# Autodesk Inventor assembly: cat
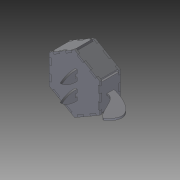
[picture p0: Inventor's stored thumbnail of the model, 180x180]
Saved by Autodesk Inventor 2015 (Build 190159000, 159)
## iProperties
Created: 2017-11-28
Part Number: cat
Document SubType Name: Assembly
Designer: Max
Author: Max
## Documents named in this file (8)
- C:\Users\Max\Dropbox\cat\cat.iam
- C:\Users\Max\Dropbox\cat\base.ipt
- C:\Users\Max\Dropbox\cat\cara.ipt
- C:\Users\Max\Dropbox\cat\lado.ipt
- C:\Users\Max\Dropbox\cat\cabeza.ipt
- C:\Users\Max\Dropbox\cat\oreja.ipt
- C:\Users\Max\Dropbox\cat\lado cola.ipt
- C:\Users\Max\Dropbox\cat\cola.ipt
## Components (11 placed, 7 different names)
1. base:1 — Flush:1, Mate:1, Mate:2, Flush:2, Mate:3, Mate:4, Flush:3, Mate:5, Mate:6, Flush:4, Mate:7, Mate:8, Flush:6, Mate:11, Mate:12, Mate:21
2. cara:1 — Flush:1, Mate:1, Mate:2, Flush:7, Mate:13, Mate:14
3. lado:1 — Flush:3, Mate:5, Mate:6
4. lado:3 — Flush:4, Mate:7, Mate:8
5. lado:5 — Flush:2, Mate:3, Mate:4
6. lado:7 — Flush:6, Mate:11, Mate:12
7. cabeza:1 — Flush:7, Mate:13, Mate:14, Mate:15, Mate:16, Mate:17, Mate:18, Mate:19, Mate:20, Flush:8, Mate:22
8. oreja:1 — Mate:18, Mate:19, Mate:20
9. oreja:2 — Mate:15, Mate:16, Mate:17
10. lado cola:1 — Flush:8, Mate:21, Mate:22, Mate:23, Mate:24
11. cola:1 — Mate:23, Mate:24
## Relationships (29: Mate 22, Flush 7)
- Flush:1: base:1 ↔ cara:1
- Mate:1: base:1 ↔ cara:1
- Mate:2: base:1 ↔ cara:1
- Flush:2: base:1 ↔ lado:5
- Mate:3: base:1 ↔ lado:5
- Mate:4: base:1 ↔ lado:5
- Flush:3: base:1 ↔ lado:1
- Mate:5: base:1 ↔ lado:1
- Mate:6: base:1 ↔ lado:1
- Flush:4: base:1 ↔ lado:3
- Mate:7: base:1 ↔ lado:3
- Mate:8: base:1 ↔ lado:3
- Flush:6: base:1 ↔ lado:7
- Mate:11: base:1 ↔ lado:7
- Mate:12: base:1 ↔ lado:7
- Flush:7: cara:1 ↔ cabeza:1
- Mate:13: cara:1 ↔ cabeza:1
- Mate:14: cara:1 ↔ cabeza:1
- Mate:15: cabeza:1 ↔ oreja:2
- Mate:16: cabeza:1 ↔ oreja:2
- Mate:17: cabeza:1 ↔ oreja:2
- Mate:18: cabeza:1 ↔ oreja:1
- Mate:19: cabeza:1 ↔ oreja:1
- Mate:20: cabeza:1 ↔ oreja:1
- Flush:8: cabeza:1 ↔ lado cola:1
- Mate:21: base:1 ↔ lado cola:1
- Mate:22: cabeza:1 ↔ lado cola:1
- Mate:23: lado cola:1 ↔ cola:1
- Mate:24: lado cola:1 ↔ cola:1
